# Autodesk Inventor assembly: транспортер
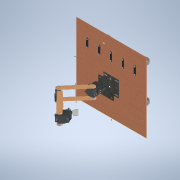
[picture p0: Inventor's stored thumbnail of the model, 180x180]
Saved by Autodesk Inventor 2020.1 (Build 241239000, 239)
## iProperties
Created: 2021-10-28
Part Number: транспортер
Document SubType Name: Assembly
Designer: Ni3na
Author: Ni3na
## Documents named in this file (10)
- C:\Users\Ni3na\Documents\GitHub\avatar-kvantoriada\3D\транспортер.iam
- C:\Users\Ni3na\Documents\GitHub\avatar-kvantoriada\3D\фанера.ipt
- C:\Users\Ni3na\Documents\GitHub\avatar-kvantoriada\3D\часть транспортера.ipt
- C:\Users\Ni3na\Documents\GitHub\avatar-kvantoriada\3D\колесо.ipt
- C:\Users\Ni3na\Documents\GitHub\avatar-kvantoriada\3D\манипулятор3.iam
- C:\Users\Ni3na\Documents\GitHub\avatar-kvantoriada\3D\магнит 2.ipt
- C:\Users\Ni3na\Documents\Inventor\Content Center Files\R2020\ru-RU\BS 4183(1)\BS 4183 - M3(1).ipt
- C:\Users\Ni3na\Documents\Inventor\Content Center Files\R2020\ru-RU\BS 4183(4)\BS 4183 - M4 x 8(1) III.ipt
- C:\Users\Ni3na\Documents\Inventor\Content Center Files\R2020\ru-RU\BS 4183(1)\BS 4183 - M4(1).ipt
- C:\Users\Ni3na\Documents\Inventor\Content Center Files\R2020\ru-RU\BS 4183(4)\BS 4183 - M3 x 8(1) III.ipt
## Components (48 placed, 9 different names)
1. фанера:1 — Жесткий:1, Жесткий:6, Жесткий:7, Жесткий:8, Жесткий:9, Жесткий:10, Жесткий:11, Жесткий:20, Жесткий:21, Жесткий:22, Жесткий:23, Жесткий:24, Жесткий:25, Жесткий:26, Жесткий:27, Жесткий:38, Жесткий:39, Жесткий:40, Жесткий:41, С поворотом:1, Жесткий:42, Жесткий:43, Жесткий:44, Жесткий:45, Жесткий:46
2. часть транспортера:1 — Жесткий:1, Жесткий:2, Жесткий:3, Жесткий:4, Жесткий:5
3. колесо:2 — Жесткий:3
4. колесо:3 — Жесткий:4
5. колесо:4 — Жесткий:5
6. колесо:5 — Жесткий:2
7. манипулятор3:1 [sub-assembly] — Жесткий:6, Жесткий:12, Жесткий:13, Жесткий:14, Жесткий:15, Жесткий:16, Жесткий:17, Жесткий:18, Жесткий:19
8. магнит 2:1 — Жесткий:11, Жесткий:36, Жесткий:37
9. магнит 2:2 — Жесткий:10, Жесткий:34, Жесткий:35
10. магнит 2:3 — Жесткий:9, Жесткий:32, Жесткий:33
11. магнит 2:4 — Жесткий:8, Жесткий:30, Жесткий:31
12. магнит 2:5 — Жесткий:7, Жесткий:28, Жесткий:29
13. BS 4183 Винты и гайки крепежные мелкие. Метрическая серия - метрическая M3 x 8:4 — Жесткий:19
14. BS 4183 Винты и гайки крепежные мелкие. Метрическая серия - метрическая M3 x 8:5 — Жесткий:12
15. BS 4183 Винты и гайки крепежные мелкие. Метрическая серия - метрическая M3 x 8:6 — Жесткий:13
16. BS 4183 Винты и гайки крепежные мелкие. Метрическая серия - метрическая M3 x 8:3 — Жесткий:18
17. BS 4183 Винты и гайки крепежные мелкие. Метрическая серия - метрическая M3 x 8:2 — Жесткий:17
18. BS 4183 Винты и гайки крепежные мелкие. Метрическая серия - метрическая M3 x 8:1 — Жесткий:16
19. BS 4183 Винты и гайки крепежные мелкие. Метрическая серия - метрическая M3 x 8:7 — Жесткий:15
20. BS 4183 Винты и гайки крепежные мелкие. Метрическая серия - метрическая M3 x 8:8 — Жесткий:14
21. BS 4183 - метрическая M3:1 — Жесткий:25
22. BS 4183 - метрическая M3:2 — Жесткий:20
23. BS 4183 - метрическая M3:3 — Жесткий:22
24. BS 4183 - метрическая M3:4 — Жесткий:24
25. BS 4183 - метрическая M3:5 — Жесткий:21
26. BS 4183 - метрическая M3:6 — Жесткий:27
27. BS 4183 - метрическая M3:7 — Жесткий:23
28. BS 4183 - метрическая M3:8 — Жесткий:26
29. BS 4183 Винты и гайки крепежные мелкие. Метрическая серия - метрическая M4 x 8:6 — Жесткий:33
30. BS 4183 Винты и гайки крепежные мелкие. Метрическая серия - метрическая M4 x 8:5 — Жесткий:32
31. BS 4183 Винты и гайки крепежные мелкие. Метрическая серия - метрическая M4 x 8:9 — Жесткий:36
32. BS 4183 Винты и гайки крепежные мелкие. Метрическая серия - метрическая M4 x 8:3 — Жесткий:30
33. BS 4183 Винты и гайки крепежные мелкие. Метрическая серия - метрическая M4 x 8:2 — Жесткий:28
34. BS 4183 Винты и гайки крепежные мелкие. Метрическая серия - метрическая M4 x 8:7 — Жесткий:34
35. BS 4183 Винты и гайки крепежные мелкие. Метрическая серия - метрическая M4 x 8:4 — Жесткий:31
36. BS 4183 Винты и гайки крепежные мелкие. Метрическая серия - метрическая M4 x 8:8 — Жесткий:35
37. BS 4183 Винты и гайки крепежные мелкие. Метрическая серия - метрическая M4 x 8:1 — Жесткий:29
38. BS 4183 Винты и гайки крепежные мелкие. Метрическая серия - метрическая M4 x 8:10 — Жесткий:37
39. BS 4183 - метрическая M4:1 — Жесткий:38
40. BS 4183 - метрическая M4:2 — Жесткий:39
41. BS 4183 - метрическая M4:3 — Жесткий:40
42. BS 4183 - метрическая M4:4 — Жесткий:41
43. BS 4183 - метрическая M4:5 — С поворотом:1
44. BS 4183 - метрическая M4:6 — Жесткий:42
45. BS 4183 - метрическая M4:7 — Жесткий:43
46. BS 4183 - метрическая M4:8 — Жесткий:46
47. BS 4183 - метрическая M4:9 — Жесткий:45
48. BS 4183 - метрическая M4:10 — Жесткий:44
## Relationships (47: WeldJoint 46, RevoluteJoint 1)
- Жесткий:1 [WeldJoint] (5 mm): фанера:1 ↔ часть транспортера:1
- Жесткий:2 [WeldJoint]: часть транспортера:1 ↔ колесо:5
- Жесткий:3 [WeldJoint]: часть транспортера:1 ↔ колесо:2
- Жесткий:4 [WeldJoint]: часть транспортера:1 ↔ колесо:3
- Жесткий:5 [WeldJoint]: часть транспортера:1 ↔ колесо:4
- Жесткий:6 [WeldJoint]: фанера:1 ↔ манипулятор3:1
- Жесткий:7 [WeldJoint]: фанера:1 ↔ магнит 2:5
- Жесткий:8 [WeldJoint]: фанера:1 ↔ магнит 2:4
- Жесткий:9 [WeldJoint]: фанера:1 ↔ магнит 2:3
- Жесткий:10 [WeldJoint]: фанера:1 ↔ магнит 2:2
- Жесткий:11 [WeldJoint]: фанера:1 ↔ магнит 2:1
- Жесткий:12 [WeldJoint]: манипулятор3:1 ↔ BS 4183 Винты и гайки крепежные мелкие. Метрическая серия - метрическая M3 x 8:5
- Жесткий:13 [WeldJoint]: манипулятор3:1 ↔ BS 4183 Винты и гайки крепежные мелкие. Метрическая серия - метрическая M3 x 8:6
- Жесткий:14 [WeldJoint]: манипулятор3:1 ↔ BS 4183 Винты и гайки крепежные мелкие. Метрическая серия - метрическая M3 x 8:8
- Жесткий:15 [WeldJoint]: манипулятор3:1 ↔ BS 4183 Винты и гайки крепежные мелкие. Метрическая серия - метрическая M3 x 8:7
- Жесткий:16 [WeldJoint]: манипулятор3:1 ↔ BS 4183 Винты и гайки крепежные мелкие. Метрическая серия - метрическая M3 x 8:1
- Жесткий:17 [WeldJoint]: манипулятор3:1 ↔ BS 4183 Винты и гайки крепежные мелкие. Метрическая серия - метрическая M3 x 8:2
- Жесткий:18 [WeldJoint]: манипулятор3:1 ↔ BS 4183 Винты и гайки крепежные мелкие. Метрическая серия - метрическая M3 x 8:3
- Жесткий:19 [WeldJoint]: манипулятор3:1 ↔ BS 4183 Винты и гайки крепежные мелкие. Метрическая серия - метрическая M3 x 8:4
- Жесткий:20 [WeldJoint]: фанера:1 ↔ BS 4183 - метрическая M3:2
- Жесткий:21 [WeldJoint]: фанера:1 ↔ BS 4183 - метрическая M3:5
- Жесткий:22 [WeldJoint]: фанера:1 ↔ BS 4183 - метрическая M3:3
- Жесткий:23 [WeldJoint]: фанера:1 ↔ BS 4183 - метрическая M3:7
- Жесткий:24 [WeldJoint]: фанера:1 ↔ BS 4183 - метрическая M3:4
- Жесткий:25 [WeldJoint]: фанера:1 ↔ BS 4183 - метрическая M3:1
- Жесткий:26 [WeldJoint]: фанера:1 ↔ BS 4183 - метрическая M3:8
- Жесткий:27 [WeldJoint]: фанера:1 ↔ BS 4183 - метрическая M3:6
- Жесткий:28 [WeldJoint]: магнит 2:5 ↔ BS 4183 Винты и гайки крепежные мелкие. Метрическая серия - метрическая M4 x 8:2
- Жесткий:29 [WeldJoint]: магнит 2:5 ↔ BS 4183 Винты и гайки крепежные мелкие. Метрическая серия - метрическая M4 x 8:1
- Жесткий:30 [WeldJoint]: магнит 2:4 ↔ BS 4183 Винты и гайки крепежные мелкие. Метрическая серия - метрическая M4 x 8:3
- Жесткий:31 [WeldJoint]: магнит 2:4 ↔ BS 4183 Винты и гайки крепежные мелкие. Метрическая серия - метрическая M4 x 8:4
- Жесткий:32 [WeldJoint]: магнит 2:3 ↔ BS 4183 Винты и гайки крепежные мелкие. Метрическая серия - метрическая M4 x 8:5
- Жесткий:33 [WeldJoint]: магнит 2:3 ↔ BS 4183 Винты и гайки крепежные мелкие. Метрическая серия - метрическая M4 x 8:6
- Жесткий:34 [WeldJoint]: магнит 2:2 ↔ BS 4183 Винты и гайки крепежные мелкие. Метрическая серия - метрическая M4 x 8:7
- Жесткий:35 [WeldJoint]: магнит 2:2 ↔ BS 4183 Винты и гайки крепежные мелкие. Метрическая серия - метрическая M4 x 8:8
- Жесткий:36 [WeldJoint]: магнит 2:1 ↔ BS 4183 Винты и гайки крепежные мелкие. Метрическая серия - метрическая M4 x 8:9
- Жесткий:37 [WeldJoint]: магнит 2:1 ↔ BS 4183 Винты и гайки крепежные мелкие. Метрическая серия - метрическая M4 x 8:10
- Жесткий:38 [WeldJoint]: фанера:1 ↔ BS 4183 - метрическая M4:1
- Жесткий:39 [WeldJoint]: фанера:1 ↔ BS 4183 - метрическая M4:2
- Жесткий:40 [WeldJoint]: фанера:1 ↔ BS 4183 - метрическая M4:3
- Жесткий:41 [WeldJoint]: фанера:1 ↔ BS 4183 - метрическая M4:4
- С поворотом:1 [RevoluteJoint]: фанера:1 ↔ BS 4183 - метрическая M4:5
- Жесткий:42 [WeldJoint]: фанера:1 ↔ BS 4183 - метрическая M4:6
- Жесткий:43 [WeldJoint]: фанера:1 ↔ BS 4183 - метрическая M4:7
- Жесткий:44 [WeldJoint]: фанера:1 ↔ BS 4183 - метрическая M4:10
- Жесткий:45 [WeldJoint]: фанера:1 ↔ BS 4183 - метрическая M4:9
- Жесткий:46 [WeldJoint]: фанера:1 ↔ BS 4183 - метрическая M4:8
